# Autodesk Inventor assembly: ASY HPR 320 hopper bin
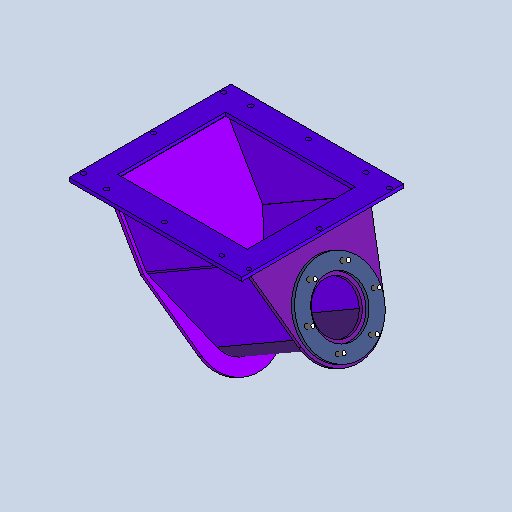
[picture p0: Inventor's stored thumbnail of the model, 512x512]
Saved by Autodesk Inventor 2025.1 (Build 291241020, 241B)
## iProperties
Created: 2025-04-01
Part Number: ASY HPR 320 hopper bin
Document SubType Name: Assembly
Designer: user
Author: user
## Documents named in this file (8)
- C:\Users\user\YandexDisk-badmisterfox\home pc\Inventor\NDM-VOS_powder_hopper\ASY HPR 320 hopper bin.iam
- C:\Users\user\YandexDisk-badmisterfox\home pc\Inventor\NDM-VOS_powder_hopper\NVPH-301 back side.ipt
- C:\Users\user\YandexDisk-badmisterfox\home pc\Inventor\NDM-VOS_powder_hopper\NVPH-306 front side.ipt
- C:\Users\user\YandexDisk-badmisterfox\home pc\Inventor\NDM-VOS_powder_hopper\ASY NVPH-466 joint flange.iam
- C:\Users\user\YandexDisk-badmisterfox\home pc\Inventor\NDM-VOS_powder_hopper\NVPH-406 second tube half.ipt
- C:\Users\user\YandexDisk-badmisterfox\home pc\Inventor\NDM-VOS_powder_hopper\NVPH-307 right side.ipt
- C:\Users\user\YandexDisk-badmisterfox\home pc\Inventor\NDM-VOS_powder_hopper\NVPH-316 main flange.ipt
- C:\Users\user\YandexDisk-badmisterfox\home pc\Inventor\NDM-VOS_powder_hopper\NVPH-307 left side.ipt
## Components (8 placed, 7 different names)
1. NVPH-301 back side:1
2. NVPH-306 front side:1
3. ASY NVPH-466 joint flange:1 [sub-assembly]
4. ASY NVPH-466 joint flange:2 [sub-assembly]
5. NVPH-406 second tube half:1
6. NVPH-307 right side:1
7. NVPH-316 main flange:1
8. NVPH-307 left side:1
## Relationships (10: WeldJoint 3, Mate 3, RevoluteJoint 2, CylindricalJoint 1, Angle 1)
- [RevoluteJoint]: NVPH-301 back side:1 ↔ ASY NVPH-466 joint flange:1
- [CylindricalJoint]: NVPH-301 back side:1 ↔ NVPH-306 front side:1
- [RevoluteJoint]: NVPH-306 front side:1 ↔ ASY NVPH-466 joint flange:2
- [WeldJoint]: NVPH-406 second tube half:1 ↔ NVPH-307 right side:1
- [WeldJoint]: NVPH-306 front side:1 ↔ NVPH-406 second tube half:1
- [Mate]: NVPH-301 back side:1 ↔ NVPH-406 second tube half:1
- [Mate]: NVPH-306 front side:1 ↔ NVPH-316 main flange:1
- [Angle] (-150 deg): NVPH-406 second tube half:1 ↔ NVPH-316 main flange:1
- [Mate]: NVPH-306 front side:1 ↔ NVPH-316 main flange:1
- [WeldJoint]: NVPH-406 second tube half:1 ↔ NVPH-307 left side:1
